# Autodesk Inventor assembly: ShortSupportPlateAssembly_MIR
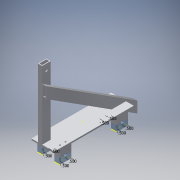
[picture p0: Inventor's stored thumbnail of the model, 180x180]
Saved by Autodesk Inventor 2016 SP1 (Build 200210100, 210)
## iProperties
Created: 2016-02-05
Part Number: ShortSupportPlateAssembly_MIR
Document SubType Name: Assembly
Designer: steele
Author: steele
## Documents named in this file (3)
- C:\snobotics\CAD-Development\robSteele\SnoBotics2016\2016-01-31-Lift\ShortSupportPlateAssembly_MIR.iam
- C:\snobotics\CAD-Development\robSteele\SnoBotics2016\2016-01-31-Lift\shortSupportPlate_MIR.ipt
- C:\snobotics\CAD-Development\robSteele\SnoBotics2016\2015-02-05-RhinoRobotNarrowView\capForLift_MIR.ipt
## Components (5 placed, 2 different names)
1. shortSupportPlate_MIR:1 — Flush:8, Flush:1, Mate:1, Flush:7, Flush:2, Mate:2, Flush:9, Flush:4, Flush:3, Mate:3, Flush:10, Flush:6, Flush:5, Mate:4
2. capForLift_MIR:1 — Flush:8, Flush:1, Mate:1
3. capForLift_MIR:2 — Flush:7, Flush:2, Mate:2
4. capForLift_MIR:3 — Flush:9, Flush:4, Flush:3, Mate:3
5. capForLift_MIR:4 — Flush:10, Flush:6, Flush:5, Mate:4
## Relationships (14: Flush 10, Mate 4)
- Flush:8: shortSupportPlate_MIR:1 ↔ capForLift_MIR:1
- Flush:1: shortSupportPlate_MIR:1 ↔ capForLift_MIR:1
- Mate:1: shortSupportPlate_MIR:1 ↔ capForLift_MIR:1
- Flush:7: shortSupportPlate_MIR:1 ↔ capForLift_MIR:2
- Flush:2: shortSupportPlate_MIR:1 ↔ capForLift_MIR:2
- Mate:2: shortSupportPlate_MIR:1 ↔ capForLift_MIR:2
- Flush:9: shortSupportPlate_MIR:1 ↔ capForLift_MIR:3
- Flush:4: shortSupportPlate_MIR:1 ↔ capForLift_MIR:3
- Flush:3: shortSupportPlate_MIR:1 ↔ capForLift_MIR:3
- Mate:3: shortSupportPlate_MIR:1 ↔ capForLift_MIR:3
- Flush:10: shortSupportPlate_MIR:1 ↔ capForLift_MIR:4
- Flush:6: shortSupportPlate_MIR:1 ↔ capForLift_MIR:4
- Flush:5: shortSupportPlate_MIR:1 ↔ capForLift_MIR:4
- Mate:4: shortSupportPlate_MIR:1 ↔ capForLift_MIR:4
